# Autodesk Inventor assembly: sweeper
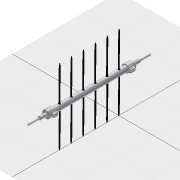
[picture p0: Inventor's stored thumbnail of the model, 180x180]
Saved by Autodesk Inventor 2015 SP1 (Build 190203100, 203)
## iProperties
Created: 2015-01-25
Part Number: sweeper
Document SubType Name: Assembly
Designer: rihoobler
Author: rihoobler
## Documents named in this file (8)
- C:\Users\datenney\Documents\GitHub\CAD\SerenityMk.2\sweeper.iam
- C:\Users\datenney\Documents\GitHub\CAD\SerenityMk.2\Sweeper tube.ipt
- C:\Users\datenney\Documents\GitHub\CAD\SerenityMk.2\Imported Components\tetrix_739077_2012\tetrix_739077_2012.ipt
- C:\Users\datenney\Documents\GitHub\CAD\SerenityMk.2\Imported Components\tetrix_739172_2012\tetrix_739172_2012.iam
- C:\Users\datenney\Documents\GitHub\CAD\SerenityMk.2\Imported Components\tetrix_739088_2012\tetrix_739088_2012.ipt
- C:\Users\datenney\Documents\GitHub\CAD\SerenityMk.2\Imported Components\tetrix_739101_2012\tetrix_739101_2012.ipt
- C:\Users\datenney\Documents\GitHub\CAD\SerenityMk.2\Imported Components\tetrix_739068_2012_288_channel\Part1.ipt
- C:\Users\datenney\Documents\GitHub\CAD\SerenityMk.2\Zip tie start.ipt
## Components (24 placed, 7 different names)
1. Sweeper tube:1 — Insert:1, Insert:2, Mate:18, Mate:19, Mate:20, Mate:21, Mate:22, Mate:23, Mate:24, Mate:25, Mate:26, Mate:27, Mate:28, Mate:29
2. tetrix_739077_2012:1 — Insert:2, Insert:4
3. tetrix_739077_2012:2 — Insert:1, Insert:3
4. tetrix_739172_2012:1 [sub-assembly] — Insert:4, Mate:15, Flush:3, Insert:7
5. tetrix_739172_2012:2 [sub-assembly] — Insert:3, Mate:16, Flush:4, Insert:5
6. tetrix_739088_2012:1 — Mate:16, Flush:4
7. tetrix_739088_2012:2 — Mate:15, Flush:3
8. tetrix_739101_2012:1 — Insert:6
9. tetrix_739101_2012:2 — Insert:5, Insert:6
10. tetrix_739101_2012:3 — Insert:8
11. tetrix_739101_2012:4 — Insert:7, Insert:8
12. Part1:1
13. Zip tie start:1 — Mate:18, Flush:10, Angle:6
14. Zip tie start:2 — Mate:22, Flush:5, Angle:1
15. Zip tie start:3 — Mate:20, Flush:7, Angle:3
16. Zip tie start:4 — Mate:19, Flush:8, Angle:4, Flush:13, Flush:14
17. Zip tie start:5 — Mate:23, Flush:9, Angle:5
18. Zip tie start:6 — Mate:21, Flush:6, Angle:2
19. Zip tie start:7 — Mate:24, Flush:10, Angle:6, Flush:15
20. Zip tie start:8 — Mate:25, Flush:9, Angle:5, Flush:14, Flush:15
21. Zip tie start:9 — Mate:26, Flush:8, Angle:4
22. Zip tie start:10 — Mate:27, Flush:7, Angle:3, Flush:12, Flush:13
23. Zip tie start:11 — Mate:28, Flush:6, Angle:2, Flush:11, Flush:12
24. Zip tie start:12 — Mate:29, Flush:5, Angle:1, Flush:11
## Relationships (41: Mate 14, Flush 13, Insert 8, Angle 6)
- Insert:1: Sweeper tube:1 ↔ tetrix_739077_2012:2
- Insert:2: Sweeper tube:1 ↔ tetrix_739077_2012:1
- Insert:3: tetrix_739077_2012:2 ↔ tetrix_739172_2012:2
- Insert:4: tetrix_739077_2012:1 ↔ tetrix_739172_2012:1
- Mate:15: tetrix_739172_2012:1 ↔ tetrix_739088_2012:2
- Flush:3 (-50.8 mm): tetrix_739172_2012:1 ↔ tetrix_739088_2012:2
- Mate:16: tetrix_739172_2012:2 ↔ tetrix_739088_2012:1
- Flush:4 (-50.8 mm): tetrix_739172_2012:2 ↔ tetrix_739088_2012:1
- Insert:5: tetrix_739172_2012:2 ↔ tetrix_739101_2012:2
- Insert:6: tetrix_739101_2012:1 ↔ tetrix_739101_2012:2
- Insert:7: tetrix_739172_2012:1 ↔ tetrix_739101_2012:4
- Insert:8: tetrix_739101_2012:3 ↔ tetrix_739101_2012:4
- Mate:18: Sweeper tube:1 ↔ Zip tie start:1
- Mate:19: Sweeper tube:1 ↔ Zip tie start:4
- Mate:20: Sweeper tube:1 ↔ Zip tie start:3
- Mate:21: Sweeper tube:1 ↔ Zip tie start:6
- Mate:22: Sweeper tube:1 ↔ Zip tie start:2
- Mate:23: Sweeper tube:1 ↔ Zip tie start:5
- Mate:24: Sweeper tube:1 ↔ Zip tie start:7
- Mate:25: Sweeper tube:1 ↔ Zip tie start:8
- Mate:26: Sweeper tube:1 ↔ Zip tie start:9
- Mate:27: Sweeper tube:1 ↔ Zip tie start:10
- Mate:28: Sweeper tube:1 ↔ Zip tie start:11
- Mate:29: Sweeper tube:1 ↔ Zip tie start:12
- Flush:5: Zip tie start:2 ↔ Zip tie start:12
- Flush:6: Zip tie start:6 ↔ Zip tie start:11
- Flush:7: Zip tie start:3 ↔ Zip tie start:10
- Flush:8: Zip tie start:4 ↔ Zip tie start:9
- Flush:9: Zip tie start:5 ↔ Zip tie start:8
- Flush:10: Zip tie start:1 ↔ Zip tie start:7
- Angle:1 (0 deg): Zip tie start:2 ↔ Zip tie start:12
- Angle:2 (0 deg): Zip tie start:6 ↔ Zip tie start:11
- Angle:3 (0 deg): Zip tie start:3 ↔ Zip tie start:10
- Angle:4 (0 deg): Zip tie start:4 ↔ Zip tie start:9
- Angle:5 (0 deg): Zip tie start:5 ↔ Zip tie start:8
- Angle:6 (0 deg): Zip tie start:1 ↔ Zip tie start:7
- Flush:11: Zip tie start:11 ↔ Zip tie start:12
- Flush:12: Zip tie start:10 ↔ Zip tie start:11
- Flush:13: Zip tie start:4 ↔ Zip tie start:10
- Flush:14: Zip tie start:4 ↔ Zip tie start:8
- Flush:15: Zip tie start:7 ↔ Zip tie start:8
